# Autodesk Inventor assembly: EnsamblajeLevitador
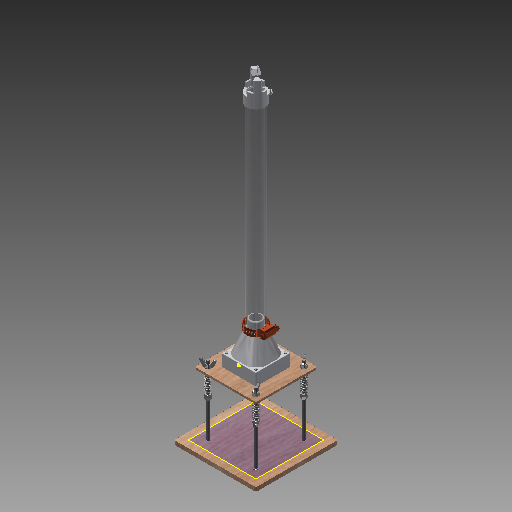
[picture p0: Inventor's stored thumbnail of the model, 512x512]
Saved by Autodesk Inventor 2017 (Build 210142000, 142)
## iProperties
Part Number: EnsamblajeLevitador
Material: Genérico
Document SubType Name: Assembly
Designer: Leonardo
Author: Leonardo
## Documents named in this file (16)
- C:\Users\Leonardo\Documents\Universidad\02 Control\Control Edgar\Laboratorio\02 Cad\EnsamblajeLevitador.iam
- C:\Users\Leonardo\Documents\Universidad\02 Control\Control Edgar\Laboratorio\02 Cad\fan80mmx20mm.iam
- C:\Users\Leonardo\Documents\Universidad\02 Control\Control Edgar\Laboratorio\02 Cad\Tubo33mmx50cm.ipt
- C:\Users\Leonardo\Documents\Universidad\02 Control\Control Edgar\Laboratorio\02 Cad\TolvaReductora.ipt
- C:\Users\Leonardo\Documents\Universidad\02 Control\Control Edgar\Laboratorio\02 Cad\TablaSoporte1.ipt
- C:\Users\Leonardo\Documents\Universidad\02 Control\Control Edgar\Laboratorio\02 Cad\TablaSoporte2.ipt
- C:\Users\Leonardo\Documents\Universidad\02 Control\Control Edgar\Laboratorio\02 Cad\TrnlloSinFin.ipt
- C:\Users\Leonardo\Documents\Universidad\02 Control\Control Edgar\Laboratorio\02 Cad\Resorte.ipt
- C:\Users\Leonardo\Documents\Universidad\02 Control\Control Edgar\Laboratorio\02 Cad\SoporteSensor.ipt
- C:\Users\Leonardo\Documents\Universidad\02 Control\Control Edgar\Laboratorio\02 Cad\SensorCJMCU530.ipt
- C:\Users\Leonardo\Documents\Inventor\Content Center Files\R2017\es-ES\ANSI B18.17(12)\ANSI B18.17 - 1_4 - 20 NormalA (1).ipt
- C:\Users\Leonardo\Documents\Inventor\Content Center Files\R2017\es-ES\AS 2465(1)\AS 2465 - 1_4  UNF(1).ipt
- C:\Users\Leonardo\Documents\Inventor\Content Center Files\R2017\es-ES\ANSI B18.3(11)\ANSI B18.3 - 5-44 UNF - 2,5(23).ipt
- C:\Users\Leonardo\Documents\Inventor\Content Center Files\R2017\es-ES\AS 1112 (2)\AS 1112 - M5  Tipo 5.ipt
- C:\Users\Leonardo\Documents\Inventor\Content Center Files\R2017\es-ES\AS 2465(1)\AS 2465 - 1_4  UNC(1).ipt
- C:\Users\Leonardo\Documents\Universidad\02 Control\Control Edgar\Laboratorio\02 Cad\Abrazadera.ipt
## Components (37 placed, 15 different names)
1. fan80mmx20mm:1 [sub-assembly] — Coincidencia:1, Coincidencia:5, Coincidencia:34, Coincidencia:35, Coincidencia:36, Coincidencia:37
2. Tubo33mmx50cm:1 — Coincidencia:1, Coincidencia:3, Coincidencia:4, Coincidencia:42
3. TolvaReductora:1 — Coincidencia:22, Coincidencia:23, Coincidencia:24, Coincidencia:25, Coincidencia:26, Coincidencia:27, Coincidencia:28, Coincidencia:29, Coincidencia:43
4. TablaSoporte1:1 — Nivelación:3, Nivelación:4, Coincidencia:5, Coincidencia:10, Coincidencia:11, Coincidencia:12, Coincidencia:13
5. TablaSoporte2:1 — Nivelación:3, Nivelación:4, Nivelación:5, Nivelación:7, Nivelación:8, Nivelación:9, Nivelación:10
6. TrnlloSinFin:1 — Nivelación:5, Coincidencia:6, Coincidencia:7, Coincidencia:8, Coincidencia:9, Coincidencia:14, Coincidencia:15, Coincidencia:16, Coincidencia:17, Coincidencia:18, Coincidencia:19, Coincidencia:20, Coincidencia:21, Coincidencia:38, Coincidencia:39, Coincidencia:40, Coincidencia:41
7. Resorte:1
8. Resorte:2
9. Resorte:3
10. Resorte:4
11. SoporteSensor:1 — Coincidencia:3, Coincidencia:4, Nivelación:6
12. SensorCJMCU530:1 — Nivelación:6
13. Tipo A - Tuerca de palomilla - Pulgadas 1/4 - 20 Normal:1 — Coincidencia:8, Coincidencia:10
14. Tipo A - Tuerca de palomilla - Pulgadas 1/4 - 20 Normal:2 — Coincidencia:6, Coincidencia:12
15. Tipo A - Tuerca de palomilla - Pulgadas 1/4 - 20 Normal:3 — Coincidencia:7, Coincidencia:13
16. Tipo A - Tuerca de palomilla - Pulgadas 1/4 - 20 Normal:4 — Coincidencia:9, Coincidencia:11
17. AS 2465 - Pulgadas 1/4  UNF:1 — Coincidencia:14
18. AS 2465 - Pulgadas 1/4  UNF:2 — Coincidencia:15
19. AS 2465 - Pulgadas 1/4  UNF:3 — Coincidencia:16
20. AS 2465 - Pulgadas 1/4  UNF:4 — Coincidencia:17
21. AS 2465 - Pulgadas 1/4  UNF:5 — Coincidencia:18
22. AS 2465 - Pulgadas 1/4  UNF:6 — Coincidencia:19
23. AS 2465 - Pulgadas 1/4  UNF:7 — Coincidencia:21
24. AS 2465 - Pulgadas 1/4  UNF:8 — Coincidencia:20
25. ANSI B18.3 - Pulgadas 5-44 UNF - 2,5:1 — Coincidencia:23, Coincidencia:27, Coincidencia:33
26. ANSI B18.3 - Pulgadas 5-44 UNF - 2,5:2 — Coincidencia:25, Coincidencia:29, Coincidencia:30
27. ANSI B18.3 - Pulgadas 5-44 UNF - 2,5:3 — Coincidencia:22, Coincidencia:26, Coincidencia:32
28. ANSI B18.3 - Pulgadas 5-44 UNF - 2,5:4 — Coincidencia:24, Coincidencia:28, Coincidencia:31
29. AS 1112 (2) - Métrico M5  Tipo 5:1 — Coincidencia:30, Coincidencia:35
30. AS 1112 (2) - Métrico M5  Tipo 5:2 — Coincidencia:31, Coincidencia:36
31. AS 1112 (2) - Métrico M5  Tipo 5:3 — Coincidencia:33, Coincidencia:37
32. AS 1112 (2) - Métrico M5  Tipo 5:4 — Coincidencia:32, Coincidencia:34
33. AS 2465 - Pulgadas 1/4  UNC:1 — Coincidencia:38, Nivelación:7
34. AS 2465 - Pulgadas 1/4  UNC:2 — Coincidencia:40, Nivelación:10
35. AS 2465 - Pulgadas 1/4  UNC:3 — Coincidencia:41, Nivelación:9
36. AS 2465 - Pulgadas 1/4  UNC:4 — Coincidencia:39, Nivelación:8
37. Abrazadera:1 — Coincidencia:42, Coincidencia:43
## Relationships (50: Mate 42, Flush 8)
- Coincidencia:1 [Mate]: fan80mmx20mm:1 ↔ Tubo33mmx50cm:1
- Nivelación:3 [Flush]: TablaSoporte1:1 ↔ TablaSoporte2:1
- Nivelación:4 [Flush] (150 mm): TablaSoporte1:1 ↔ TablaSoporte2:1
- Nivelación:5 [Flush]: TablaSoporte2:1 ↔ TrnlloSinFin:1
- Coincidencia:3 [Mate]: Tubo33mmx50cm:1 ↔ SoporteSensor:1
- Coincidencia:4 [Mate]: Tubo33mmx50cm:1 ↔ SoporteSensor:1
- Nivelación:6 [Flush]: SoporteSensor:1 ↔ SensorCJMCU530:1
- Coincidencia:5 [Mate]: fan80mmx20mm:1 ↔ TablaSoporte1:1
- Coincidencia:6 [Mate]: TrnlloSinFin:1 ↔ Tipo A - Tuerca de palomilla - Pulgadas 1/4 - 20 Normal:2
- Coincidencia:7 [Mate]: TrnlloSinFin:1 ↔ Tipo A - Tuerca de palomilla - Pulgadas 1/4 - 20 Normal:3
- Coincidencia:8 [Mate]: TrnlloSinFin:1 ↔ Tipo A - Tuerca de palomilla - Pulgadas 1/4 - 20 Normal:1
- Coincidencia:9 [Mate]: TrnlloSinFin:1 ↔ Tipo A - Tuerca de palomilla - Pulgadas 1/4 - 20 Normal:4
- Coincidencia:10 [Mate]: TablaSoporte1:1 ↔ Tipo A - Tuerca de palomilla - Pulgadas 1/4 - 20 Normal:1
- Coincidencia:11 [Mate]: TablaSoporte1:1 ↔ Tipo A - Tuerca de palomilla - Pulgadas 1/4 - 20 Normal:4
- Coincidencia:12 [Mate]: TablaSoporte1:1 ↔ Tipo A - Tuerca de palomilla - Pulgadas 1/4 - 20 Normal:2
- Coincidencia:13 [Mate]: TablaSoporte1:1 ↔ Tipo A - Tuerca de palomilla - Pulgadas 1/4 - 20 Normal:3
- Coincidencia:14 [Mate]: TrnlloSinFin:1 ↔ AS 2465 - Pulgadas 1/4  UNF:1
- Coincidencia:15 [Mate]: TrnlloSinFin:1 ↔ AS 2465 - Pulgadas 1/4  UNF:2
- Coincidencia:16 [Mate]: TrnlloSinFin:1 ↔ AS 2465 - Pulgadas 1/4  UNF:3
- Coincidencia:17 [Mate]: TrnlloSinFin:1 ↔ AS 2465 - Pulgadas 1/4  UNF:4
- Coincidencia:18 [Mate]: TrnlloSinFin:1 ↔ AS 2465 - Pulgadas 1/4  UNF:5
- Coincidencia:19 [Mate]: TrnlloSinFin:1 ↔ AS 2465 - Pulgadas 1/4  UNF:6
- Coincidencia:20 [Mate]: TrnlloSinFin:1 ↔ AS 2465 - Pulgadas 1/4  UNF:8
- Coincidencia:21 [Mate]: TrnlloSinFin:1 ↔ AS 2465 - Pulgadas 1/4  UNF:7
- Coincidencia:22 [Mate]: TolvaReductora:1 ↔ ANSI B18.3 - Pulgadas 5-44 UNF - 2,5:3
- Coincidencia:23 [Mate]: TolvaReductora:1 ↔ ANSI B18.3 - Pulgadas 5-44 UNF - 2,5:1
- Coincidencia:24 [Mate]: TolvaReductora:1 ↔ ANSI B18.3 - Pulgadas 5-44 UNF - 2,5:4
- Coincidencia:25 [Mate]: TolvaReductora:1 ↔ ANSI B18.3 - Pulgadas 5-44 UNF - 2,5:2
- Coincidencia:26 [Mate]: TolvaReductora:1 ↔ ANSI B18.3 - Pulgadas 5-44 UNF - 2,5:3
- Coincidencia:27 [Mate]: TolvaReductora:1 ↔ ANSI B18.3 - Pulgadas 5-44 UNF - 2,5:1
- Coincidencia:28 [Mate]: TolvaReductora:1 ↔ ANSI B18.3 - Pulgadas 5-44 UNF - 2,5:4
- Coincidencia:29 [Mate]: TolvaReductora:1 ↔ ANSI B18.3 - Pulgadas 5-44 UNF - 2,5:2
- Coincidencia:30 [Mate]: ANSI B18.3 - Pulgadas 5-44 UNF - 2,5:2 ↔ AS 1112 (2) - Métrico M5  Tipo 5:1
- Coincidencia:31 [Mate]: ANSI B18.3 - Pulgadas 5-44 UNF - 2,5:4 ↔ AS 1112 (2) - Métrico M5  Tipo 5:2
- Coincidencia:32 [Mate]: ANSI B18.3 - Pulgadas 5-44 UNF - 2,5:3 ↔ AS 1112 (2) - Métrico M5  Tipo 5:4
- Coincidencia:33 [Mate]: ANSI B18.3 - Pulgadas 5-44 UNF - 2,5:1 ↔ AS 1112 (2) - Métrico M5  Tipo 5:3
- Coincidencia:34 [Mate]: fan80mmx20mm:1 ↔ AS 1112 (2) - Métrico M5  Tipo 5:4
- Coincidencia:35 [Mate]: fan80mmx20mm:1 ↔ AS 1112 (2) - Métrico M5  Tipo 5:1
- Coincidencia:36 [Mate]: fan80mmx20mm:1 ↔ AS 1112 (2) - Métrico M5  Tipo 5:2
- Coincidencia:37 [Mate]: fan80mmx20mm:1 ↔ AS 1112 (2) - Métrico M5  Tipo 5:3
- Coincidencia:38 [Mate]: TrnlloSinFin:1 ↔ AS 2465 - Pulgadas 1/4  UNC:1
- Coincidencia:39 [Mate]: TrnlloSinFin:1 ↔ AS 2465 - Pulgadas 1/4  UNC:4
- Coincidencia:40 [Mate]: TrnlloSinFin:1 ↔ AS 2465 - Pulgadas 1/4  UNC:2
- Coincidencia:41 [Mate]: TrnlloSinFin:1 ↔ AS 2465 - Pulgadas 1/4  UNC:3
- Nivelación:7 [Flush]: TablaSoporte2:1 ↔ AS 2465 - Pulgadas 1/4  UNC:1
- Nivelación:8 [Flush]: TablaSoporte2:1 ↔ AS 2465 - Pulgadas 1/4  UNC:4
- Nivelación:9 [Flush]: TablaSoporte2:1 ↔ AS 2465 - Pulgadas 1/4  UNC:3
- Nivelación:10 [Flush]: TablaSoporte2:1 ↔ AS 2465 - Pulgadas 1/4  UNC:2
- Coincidencia:42 [Mate]: Tubo33mmx50cm:1 ↔ Abrazadera:1
- Coincidencia:43 [Mate]: TolvaReductora:1 ↔ Abrazadera:1
